# Autodesk Inventor assembly: assembly
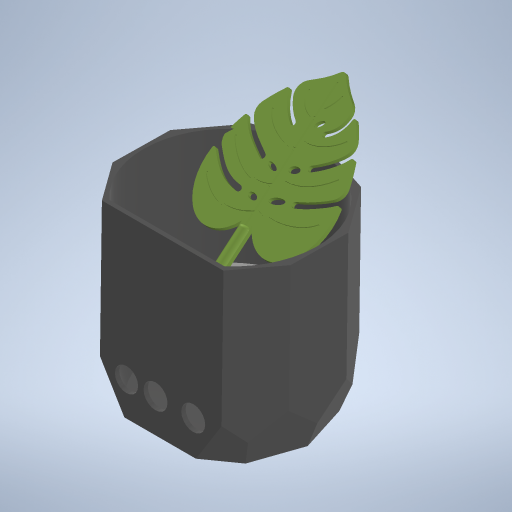
[picture p0: Inventor's stored thumbnail of the model, 512x512]
Saved by Autodesk Inventor 2024.2 (Build 282272000, 272)
## iProperties
Created: 2024-04-10
Part Number: assembly
Document SubType Name: Assembly
Designer: Micha
Author: Micha
## Documents named in this file (4)
- C:\Users\Micha\Documents\493\a1\assembly.iam
- C:\Users\Micha\Documents\493\a1\Cover.ipt
- C:\Users\Micha\Documents\493\a1\Leaf.ipt
- C:\Users\Micha\Documents\493\a1\Vase.ipt
## Components (3 placed, 3 different names)
1. Cover:1 — Insert:1, Mate:1, Mate:2
2. Leaf:1 — Mate:2
3. Vase:1 — Insert:1, Mate:1
## Relationships (3: Mate 2, Insert 1)
- Insert:1: Cover:1 ↔ Vase:1
- Mate:1: Cover:1 ↔ Vase:1
- Mate:2: Cover:1 ↔ Leaf:1
